# Autodesk Inventor assembly: nanotwister_reaper
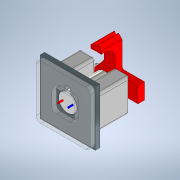
[picture p0: Inventor's stored thumbnail of the model, 180x180]
Saved by Autodesk Inventor 2021 (Build 250183000, 183)
## iProperties
Created: 2022-02-27
Part Number: nanotwister_reaper
Document SubType Name: Assembly
Designer: ermoz
Author: ermoz
## Documents named in this file (10)
- D:\Moje Wyczyny\My_Poor_Projects\nanosumo-nanotwister\mechanics\nanotwister_reaper.iam
- D:\Moje Wyczyny\My_Poor_Projects\nanosumo-nanotwister\mechanics\motor_noname.ipt
- D:\Moje Wyczyny\My_Poor_Projects\nanosumo-nanotwister\mechanics\pb_hole.ipt
- D:\Moje Wyczyny\My_Poor_Projects\nanosumo-nanotwister\mechanics\hot_glue_mashroom.ipt
- D:\Moje Wyczyny\My_Poor_Projects\nanosumo-nanotwister\mechanics\battery_1S_100mAh_no_prot.ipt
- D:\Moje Wyczyny\My_Poor_Projects\nanosumo-nanotwister\mechanics\rotor_core.ipt
- D:\Moje Wyczyny\My_Poor_Projects\nanosumo-nanotwister\mechanics\3M_Nut.ipt
- D:\Moje Wyczyny\My_Poor_Projects\nanosumo-nanotwister\mechanics\wire.ipt
- D:\Moje Wyczyny\My_Poor_Projects\nanosumo-nanotwister\mechanics\metal_connector.ipt
- D:\Moje Wyczyny\My_Poor_Projects\nanosumo-nanotwister\mechanics\connector_screw.ipt
## Components (14 placed, 9 different names)
1. motor_noname:1 — Mate:1, Mate:5, Tangent:1, Tangent:2, Tangent:9, Angle:5, Tangent:10, Mate:20, Tangent:11
2. pb_hole:1 — Mate:1, Mate:4, Flush:2, Flush:3, Mate:6, Mate:7, Angle:1, Angle:2, Angle:8
3. hot_glue_mashroom:1 — Mate:4, Flush:2, Flush:3, Mate:5
4. battery_1S_100mAh_no_prot:1 — Mate:6, Tangent:1, Angle:1
5. battery_1S_100mAh_no_prot:2 — Mate:7, Tangent:2, Angle:2
6. rotor_core:1 — Mate:23, Angle:9, Mate:24
7. 3M_Nut:1 — Mate:16
8. 3M_Nut:2 — Mate:16
9. 3M_Nut:3 — Mate:15
10. 3M_Nut:4 — Mate:15
11. wire:1
12. wire:2
13. metal_connector:1 — Mate:19, Tangent:9, Angle:5, Mate:20, Mate:21, Angle:9, Mate:24, Angle:10
14. connector_screw:1 — Mate:19, Tangent:10, Mate:21, Mate:23
## Relationships (25: Mate 12, Angle 6, Tangent 5, Flush 2)
- Mate:1: motor_noname:1 ↔ pb_hole:1
- Mate:4: pb_hole:1 ↔ hot_glue_mashroom:1
- Flush:2 (0.25 mm): pb_hole:1 ↔ hot_glue_mashroom:1
- Flush:3 (0.25 mm): pb_hole:1 ↔ hot_glue_mashroom:1
- Mate:5: motor_noname:1 ↔ hot_glue_mashroom:1
- Mate:6: pb_hole:1 ↔ battery_1S_100mAh_no_prot:1
- Mate:7: pb_hole:1 ↔ battery_1S_100mAh_no_prot:2
- Tangent:1: motor_noname:1 ↔ battery_1S_100mAh_no_prot:1
- Tangent:2: motor_noname:1 ↔ battery_1S_100mAh_no_prot:2
- Angle:1 (0 deg): pb_hole:1 ↔ battery_1S_100mAh_no_prot:1
- Angle:2 (0 deg): pb_hole:1 ↔ battery_1S_100mAh_no_prot:2
- Mate:15: 3M_Nut:3 ↔ 3M_Nut:4
- Mate:16: 3M_Nut:1 ↔ 3M_Nut:2
- Mate:19: metal_connector:1 ↔ connector_screw:1
- Tangent:9: motor_noname:1 ↔ metal_connector:1
- Angle:5 (0 deg): motor_noname:1 ↔ metal_connector:1
- Tangent:10: motor_noname:1 ↔ connector_screw:1
- Mate:20 (0.5 mm): motor_noname:1 ↔ metal_connector:1
- Mate:21 (1.6 mm): metal_connector:1 ↔ connector_screw:1
- Mate:23: rotor_core:1 ↔ connector_screw:1
- Angle:8 (0 deg): pb_hole:1
- Angle:9 (0 deg): rotor_core:1 ↔ metal_connector:1
- Mate:24 (0.2 mm): rotor_core:1 ↔ metal_connector:1
- Angle:10 (0 deg): metal_connector:1
- Tangent:11 (0.4 mm): motor_noname:1
